# Autodesk Inventor assembly: Poste de travail_MIR2
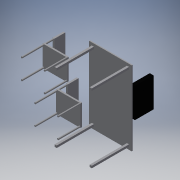
[picture p0: Inventor's stored thumbnail of the model, 180x180]
Saved by Autodesk Inventor 2016 SP1 (Build 200210100, 210)
## iProperties
Created: 2016-10-04
Part Number: Poste de travail_MIR2
Material: Générique
Document SubType Name: Assembly
Designer: dimercur
Author: dimercur
EcartPiedChaise: 100,000 mm
ChaiseAvancée: 300,000 mm
ChaiseReculée: 550,000 mm
## Documents named in this file (4)
- D:\Users\dimercur\Documents\SVN\projets-gei\Salle 22-24\Poste de travail_MIR2.iam
- D:\Users\dimercur\Documents\SVN\projets-gei\Salle 22-24\Chaise_MIR2.ipt
- D:\Users\dimercur\Documents\SVN\projets-gei\Salle 22-24\Table_MIR2.ipt
- D:\Users\dimercur\Documents\SVN\projets-gei\Salle 22-24\Ecran_MIR1.ipt
## Components (4 placed, 3 different names)
1. Chaise_MIR2:1 — Placage:3, Placage:2, Affleurement:1
2. Chaise_MIR2:2 — Placage:4, Affleurement:2, Placage:1
3. Table_MIR2:1 — Placage:4, Placage:3, Placage:2, Affleurement:2, Affleurement:1, Placage:1, Placage:6, Placage:5
4. Ecran_MIR1:1 — Placage:6, Placage:5
## Relationships (8: Mate 6, Flush 2)
- Placage:4 [Mate] (550 mm): Chaise_MIR2:2 ↔ Table_MIR2:1
- Placage:3 [Mate] (300 mm): Chaise_MIR2:1 ↔ Table_MIR2:1
- Placage:2 [Mate] (100 mm): Chaise_MIR2:1 ↔ Table_MIR2:1
- Affleurement:2 [Flush]: Chaise_MIR2:2 ↔ Table_MIR2:1
- Affleurement:1 [Flush]: Chaise_MIR2:1 ↔ Table_MIR2:1
- Placage:1 [Mate] (100 mm): Chaise_MIR2:2 ↔ Table_MIR2:1
- Placage:6 [Mate] (50 mm): Table_MIR2:1 ↔ Ecran_MIR1:1
- Placage:5 [Mate]: Table_MIR2:1 ↔ Ecran_MIR1:1
